# Autodesk Inventor assembly: Tetrix_739197
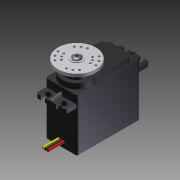
[picture p0: Inventor's stored thumbnail of the model, 180x180]
Saved by Autodesk Inventor 2015 SP1 (Build 190203100, 203)
## iProperties
Category: Servo
Company: Autodesk Inc.
Created: 2014-11-19
Part Number: Tetrix_739197
Document SubType Name: Assembly
Designer: Tetrix
Vendor: Tetrix
Author: Autodesk Inc.
## Documents named in this file (5)
- D:\Data Folder\FTC 2015\KOP\Tetrix\Tetrix_739197.iam
- D:\Data Folder\FTC 2015\KOP\Tetrix\Tetrix_739197_Servo.ipt
- D:\Data Folder\FTC 2015\KOP\Tetrix\Tetrix_739197_Metal_Horn.ipt
- D:\Data Folder\FTC 2015\KOP\Tetrix\Tetrix_739197_Screw.ipt
- D:\Data Folder\FTC 2015\KOP\Tetrix\Tetrix_739197_Plastic_Horn.ipt
## Components (5 placed, 4 different names)
1. Tetrix_739197_Servo — Insert:1, Insert:2
2. Tetrix_739197_Metal_Horn — Insert:2, Insert:3
3. Tetrix_739197_Screw — Insert:3
4. Tetrix_739197_Plastic_Horn — Insert:1, Insert:4
5. Tetrix_739197_Screw:2 — Insert:4
## Relationships (4: Insert 4)
- Insert:1: Tetrix_739197_Servo ↔ Tetrix_739197_Plastic_Horn
- Insert:2: Tetrix_739197_Servo ↔ Tetrix_739197_Metal_Horn
- Insert:3: Tetrix_739197_Metal_Horn ↔ Tetrix_739197_Screw
- Insert:4: Tetrix_739197_Plastic_Horn ↔ Tetrix_739197_Screw:2
